# Autodesk Inventor assembly: suspension_one_side
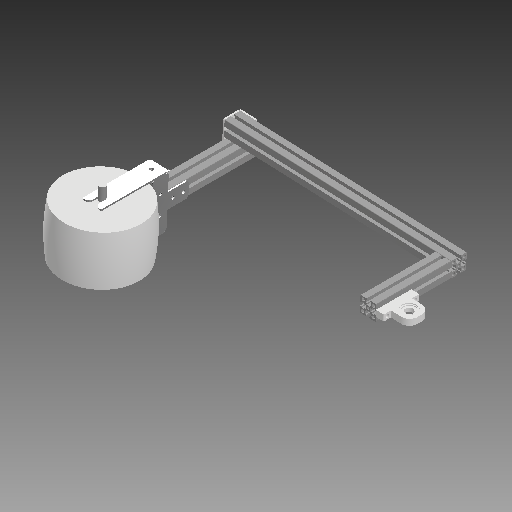
[picture p0: Inventor's stored thumbnail of the model, 512x512]
Saved by Autodesk Inventor 2021.3 (Build 253353000, 353)
## iProperties
Created: 2021-05-27
Part Number: suspension_one_side
Document SubType Name: Assembly
Designer: gisen
Author: gisen
## Documents named in this file (9)
- C:\Users\gisen\workspace\beetle_inventor_model\suspension\rocker_right.iam
- C:\Users\gisen\workspace\beetle_inventor_model\suspension\C-BGHKA6902ZZ-30\C-BGHKA6902ZZ-30.iam
- C:\Users\gisen\workspace\beetle_inventor_model\suspension\frame\AFS-3030-435.ipt
- C:\Users\gisen\workspace\beetle_inventor_model\suspension\frame\AFS-3030-200.ipt
- C:\Users\gisen\workspace\beetle_inventor_model\suspension\wheel_with_mounts.iam
- C:\Users\gisen\workspace\beetle_inventor_model\suspension\frame\AFS-3030-174.ipt
- C:\Users\gisen\workspace\beetle_inventor_model\suspension\CAM\rocker_frame_mount_00.ipt
- C:\Users\gisen\workspace\beetle_inventor_model\suspension\CAM\wheel_frame_mount.ipt
- C:\Users\gisen\workspace\beetle_inventor_model\suspension\CAM\rocker_frame_mount_01.ipt
## Components (8 placed, 8 different names)
1. C-BGHKA6902ZZ-30:1 [sub-assembly] — メイト:5, メイト:18, 角度:1, フラッシュ:15
2. AFS-3030-435:1 — メイト:5, フラッシュ:6, フラッシュ:7, メイト:6, メイト:8, メイト:15, フラッシュ:9, メイト:17, フラッシュ:11, メイト:21
3. AFS-3030-174:1 — フラッシュ:6, フラッシュ:7, メイト:6, メイト:18, 角度:1, フラッシュ:15
4. rocker_frame_mount_00:1 — メイト:8, メイト:16, メイト:17, フラッシュ:11
5. AFS-3030-200:1 — メイト:13, フラッシュ:8, メイト:14, メイト:15, フラッシュ:9, メイト:16, メイト:20, フラッシュ:14
6. wheel_with_mounts:1 [sub-assembly] — メイト:13, フラッシュ:8, メイト:14, フラッシュ:10, フラッシュ:12, フラッシュ:13, メイト:19
7. wheel_frame_mount:1 — フラッシュ:12, フラッシュ:13, メイト:19
8. rocker_frame_mount_01:1 — メイト:20, メイト:21, フラッシュ:14
## Relationships (23: Mate 12, Flush 10, Angle 1)
- メイト:5 [Mate] (-15 mm): C-BGHKA6902ZZ-30:1 ↔ AFS-3030-435:1
- フラッシュ:6 [Flush]: AFS-3030-435:1 ↔ AFS-3030-174:1
- フラッシュ:7 [Flush]: AFS-3030-435:1 ↔ AFS-3030-174:1
- メイト:6 [Mate]: AFS-3030-435:1 ↔ AFS-3030-174:1
- メイト:8 [Mate]: AFS-3030-435:1 ↔ rocker_frame_mount_00:1
- メイト:13 [Mate]: AFS-3030-200:1 ↔ wheel_with_mounts:1
- フラッシュ:8 [Flush]: AFS-3030-200:1 ↔ wheel_with_mounts:1
- メイト:14 [Mate]: AFS-3030-200:1 ↔ wheel_with_mounts:1
- メイト:15 [Mate] (3 mm): AFS-3030-435:1 ↔ AFS-3030-200:1
- フラッシュ:9 [Flush]: AFS-3030-435:1 ↔ AFS-3030-200:1
- メイト:16 [Mate]: rocker_frame_mount_00:1 ↔ AFS-3030-200:1
- メイト:17 [Mate]: AFS-3030-435:1 ↔ rocker_frame_mount_00:1
- メイト:18 [Mate]: C-BGHKA6902ZZ-30:1 ↔ AFS-3030-174:1
- フラッシュ:10 [Flush]: wheel_with_mounts:1
- フラッシュ:11 [Flush]: AFS-3030-435:1 ↔ rocker_frame_mount_00:1
- フラッシュ:12 [Flush]: wheel_with_mounts:1 ↔ wheel_frame_mount:1
- フラッシュ:13 [Flush]: wheel_with_mounts:1 ↔ wheel_frame_mount:1
- メイト:19 [Mate]: wheel_with_mounts:1 ↔ wheel_frame_mount:1
- メイト:20 [Mate]: AFS-3030-200:1 ↔ rocker_frame_mount_01:1
- メイト:21 [Mate]: AFS-3030-435:1 ↔ rocker_frame_mount_01:1
- フラッシュ:14 [Flush]: AFS-3030-200:1 ↔ rocker_frame_mount_01:1
- 角度:1 [Angle] (0 deg): C-BGHKA6902ZZ-30:1 ↔ AFS-3030-174:1
- フラッシュ:15 [Flush]: C-BGHKA6902ZZ-30:1 ↔ AFS-3030-174:1
